# Autodesk Inventor assembly: locomotion assembly
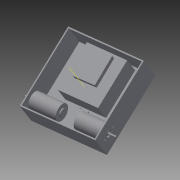
[picture p0: Inventor's stored thumbnail of the model, 180x180]
Saved by Autodesk Inventor 2015 (Build 190159000, 159)
## iProperties
Created: 2014-10-11
Part Number: locomotion assembly
Document SubType Name: Assembly
Designer: ericd_000
Author: ericd_000
## Documents named in this file (7)
- C:\Users\ericd_000\Dropbox\GitHub\initial_cad\eric_cad\locomotion assembly.iam
- C:\Users\ericd_000\Dropbox\GitHub\initial_cad\eric_cad\locomotion box.ipt
- C:\Users\ericd_000\Dropbox\GitHub\initial_cad\eric_cad\male bayonet connector 10.ipt
- C:\Users\ericd_000\Dropbox\GitHub\initial_cad\eric_cad\Imported Components\217-2000\217-2000.ipt
- C:\Users\ericd_000\Dropbox\GitHub\initial_cad\eric_cad\stark24v10ahbattery.ipt
- C:\Users\ericd_000\Dropbox\GitHub\initial_cad\eric_cad\udoo.ipt
- C:\Users\ericd_000\Dropbox\GitHub\initial_cad\eric_cad\Imported Components\M4 10mm length\M4 10mm length.ipt
## Components (10 placed, 6 different names)
1. locomotion box:1 — Mate:1, Cylindrical:1, Cylindrical:2, Mate:2, Mate:4, Cylindrical:4, Cylindrical:6, Mate:5, Mate:6, Mate:7, Cylindrical:8, Cylindrical:9, Mate:8, Mate:9, Mate:10
2. male bayonet connector 10:1 — Mate:1, Cylindrical:1, Cylindrical:2
3. 217-2000:1 — Cylindrical:10, Cylindrical:11, Mate:8
4. 217-2000:2 — Cylindrical:5, Cylindrical:7, Mate:5
5. stark24v10ahbattery:1 — Mate:2, Mate:3, Mate:4
6. udoo:1 — Mate:3
7. M4 10mm length:1 — Cylindrical:6, Cylindrical:7, Mate:7
8. M4 10mm length:2 — Cylindrical:4, Cylindrical:5, Mate:6
9. M4 10mm length:3 — Cylindrical:8, Cylindrical:11, Mate:10
10. M4 10mm length:4 — Cylindrical:9, Cylindrical:10, Mate:9
## Relationships (20: Mate 10, CylindricalJoint 10)
- Mate:1: locomotion box:1 ↔ male bayonet connector 10:1
- Cylindrical:1: locomotion box:1 ↔ male bayonet connector 10:1
- Cylindrical:2: locomotion box:1 ↔ male bayonet connector 10:1
- Mate:2 (1 mm): locomotion box:1 ↔ stark24v10ahbattery:1
- Mate:3 (2 mm): stark24v10ahbattery:1 ↔ udoo:1
- Mate:4 (10 mm): locomotion box:1 ↔ stark24v10ahbattery:1
- Cylindrical:4: locomotion box:1 ↔ M4 10mm length:2
- Cylindrical:5: 217-2000:2 ↔ M4 10mm length:2
- Cylindrical:6: locomotion box:1 ↔ M4 10mm length:1
- Cylindrical:7: 217-2000:2 ↔ M4 10mm length:1
- Mate:5 (0.1 mm): locomotion box:1 ↔ 217-2000:2
- Mate:6: locomotion box:1 ↔ M4 10mm length:2
- Mate:7: locomotion box:1 ↔ M4 10mm length:1
- Cylindrical:8: locomotion box:1 ↔ M4 10mm length:3
- Cylindrical:9: locomotion box:1 ↔ M4 10mm length:4
- Cylindrical:10: 217-2000:1 ↔ M4 10mm length:4
- Cylindrical:11: 217-2000:1 ↔ M4 10mm length:3
- Mate:8 (0.1 mm): locomotion box:1 ↔ 217-2000:1
- Mate:9: locomotion box:1 ↔ M4 10mm length:4
- Mate:10: locomotion box:1 ↔ M4 10mm length:3
